# Autodesk Inventor assembly: Assembly1
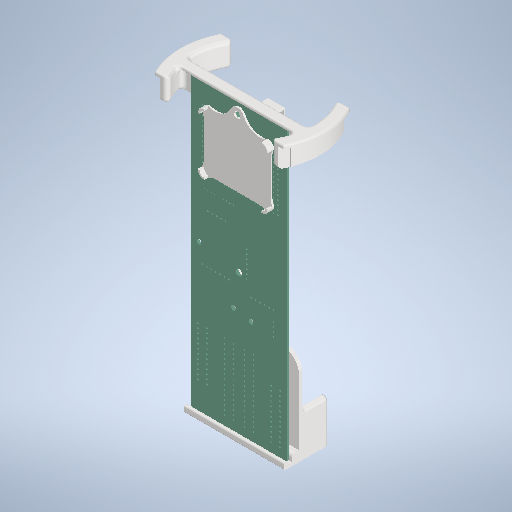
[picture p0: Inventor's stored thumbnail of the model, 512x512]
Saved by Autodesk Inventor 2025.3 (Build 293356000, 356)
## iProperties
Created: 2024-07-03
Part Number: Assembly1
Document SubType Name: Assembly
Designer: vncnt
Author: vncnt
## Documents named in this file (8)
- C:\Users\vncnt\OneDrive\Documents\Inventor\ASRC\Air Quality Sensor\Air Quality Board Mount\AQS Assembly.iam
- C:\Users\vncnt\OneDrive\Documents\Inventor\ASRC\Air Quality Sensor\Air Quality Board Mount\PVC.ipt
- C:\Users\vncnt\OneDrive\Documents\Inventor\ASRC\Air Quality Sensor\Air Quality Board Mount\CSL AQS V1 spin3.iam
- C:\Users\vncnt\OneDrive\Documents\Inventor\ASRC\Air Quality Sensor\Air Quality Board Mount\AQS Mount V6.ipt
- C:\Users\vncnt\OneDrive\Documents\Inventor\ASRC\Air Quality Sensor\Air Quality Board Mount\3in End Cap\3in End Cap.ipt
- C:\Users\vncnt\OneDrive\Documents\Inventor\ASRC\Air Quality Sensor\Air Quality Board Mount\SEN5X Mount V4.ipt
- C:\Users\vncnt\OneDrive\Documents\Inventor\ASRC\Air Quality Sensor\Air Quality Board Mount\Solar Board Mount V1.ipt
- C:\Users\vncnt\OneDrive\Documents\Inventor\ASRC\Air Quality Sensor\Air Quality Board Mount\Battery Mount V1.ipt
## Components (7 placed, 7 different names)
1. PVC:1 — Mate:1, Mate:2, Flush:1, Mate:3, Mate:4, Mate:5, Flush:2, Mate:16
2. CSL AQS V1 spin3:1 [sub-assembly] — Mate:5, Mate:7, Mate:9, Mate:11, Mate:15, Mate:17, Mate:18
3. 3in End Cap:1 — Mate:3, Mate:4
4. AQS Mount V6:1 — Mate:7, Flush:2, Mate:15, Mate:16, Angle:1, Mate:19, Mate:20
5. SEN5X Mount V4:1 — Mate:9, Mate:11, Mate:21
6. Solar Board Mount V1:1 — Mate:17, Mate:18, Angle:1
7. Battery Mount V1:1 — Mate:19, Mate:20, Mate:21
## Relationships (18: Mate 15, Flush 2, Angle 1)
- Mate:1: PVC:1
- Mate:2: PVC:1
- Flush:1: PVC:1
- Mate:3: PVC:1 ↔ 3in End Cap:1
- Mate:4: PVC:1 ↔ 3in End Cap:1
- Mate:5: PVC:1 ↔ CSL AQS V1 spin3:1
- Mate:7: CSL AQS V1 spin3:1 ↔ AQS Mount V6:1
- Flush:2: PVC:1 ↔ AQS Mount V6:1
- Mate:9: CSL AQS V1 spin3:1 ↔ SEN5X Mount V4:1
- Mate:11: CSL AQS V1 spin3:1 ↔ SEN5X Mount V4:1
- Mate:15: CSL AQS V1 spin3:1 ↔ AQS Mount V6:1
- Mate:16: PVC:1 ↔ AQS Mount V6:1
- Mate:17: CSL AQS V1 spin3:1 ↔ Solar Board Mount V1:1
- Mate:18: CSL AQS V1 spin3:1 ↔ Solar Board Mount V1:1
- Angle:1 (90 deg): AQS Mount V6:1 ↔ Solar Board Mount V1:1
- Mate:19: AQS Mount V6:1 ↔ Battery Mount V1:1
- Mate:20: AQS Mount V6:1 ↔ Battery Mount V1:1
- Mate:21: SEN5X Mount V4:1 ↔ Battery Mount V1:1
